# Autodesk Inventor assembly: Elbow
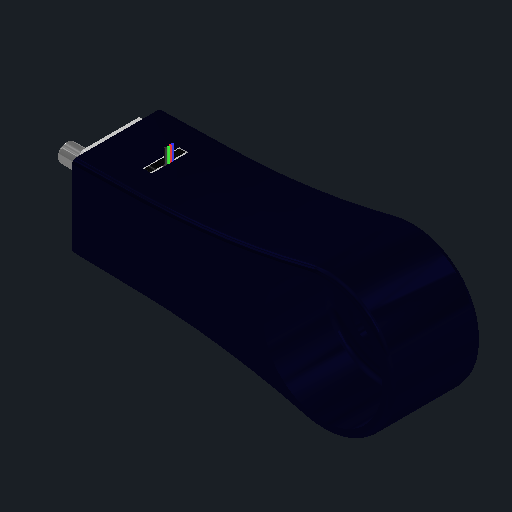
[picture p0: Inventor's stored thumbnail of the model, 512x512]
Saved by Autodesk Inventor 2023 (Build 270158000, 158)
## iProperties
Created: 2023-04-09
Part Number: Elbow
Document SubType Name: Assembly
Designer: vatdu
Author: vatdu
## Documents named in this file (3)
- C:\Users\vatdu\Desktop\CRYSTAL MARK II\Arm\Elbow\Elbow.iam
- C:\Users\vatdu\Desktop\CRYSTAL MARK II\Arm\Elbow\Arm.ipt
- C:\Users\vatdu\Desktop\CRYSTAL MARK II\Components\Stepper Motor.ipt
## Components (2 placed, 2 different names)
1. Arm:1 — Rigid:1
2. Stepper Motor:1 — Rigid:1
## Relationships (1: WeldJoint 1)
- Rigid:1 [WeldJoint]: Arm:1 ↔ Stepper Motor:1
